# Autodesk Inventor assembly: Structure
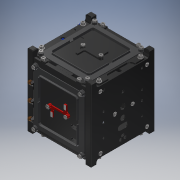
[picture p0: Inventor's stored thumbnail of the model, 180x180]
Saved by Autodesk Inventor 2018 (Build 220112000, 112)
## iProperties
Created: 2019-03-30
Part Number: Structure
Document SubType Name: Assembly
Designer: Bradley
Author: Bradley
## Documents named in this file (19)
- C:\Users\Bradley\Documents\GitHub\CougSat1-Hardware\CougSat1-Structure\CADModel\Imported\Structure.iam
- C:\Users\Bradley\Documents\GitHub\CougSat1-Hardware\CougSat1-Structure\CADModel\Imported\Structure_+X.ipt
- C:\Users\Bradley\Documents\GitHub\CougSat1-Hardware\CougSat1-Structure\CADModel\Imported\Structure_-X.ipt
- C:\Users\Bradley\Documents\GitHub\CougSat1-Hardware\CougSat1-Structure\CADModel\Imported\Structure_Y.ipt
- C:\Users\Bradley\Documents\GitHub\CougSat1-Hardware\CougSat1-Structure\CADModel\Imported\Structure_-Z.ipt
- C:\Users\Bradley\Documents\GitHub\CougSat1-Hardware\CougSat1-Structure\CADModel\Imported\Structure_SolarPanelHeatsink.ipt
- C:\Users\Bradley\Documents\GitHub\CougSat1-Hardware\CougSat1-Structure\CADModel\Imported\Structure_MagnetorquerForm.ipt
- C:\Users\Bradley\Documents\GitHub\Resources\SupplierDocuments\48 - Hardware\48-0361\48-0361.ipt
- C:\Users\Bradley\Documents\GitHub\Resources\SupplierDocuments\48 - Hardware\48-0340\48-0340.ipt
- C:\Users\Bradley\Documents\GitHub\Resources\SupplierDocuments\48 - Hardware\48-0350\48-0350.ipt
- C:\Users\Bradley\Documents\GitHub\Resources\SupplierDocuments\48 - Hardware\48-0300\48-0300.ipt
- C:\Users\Bradley\Documents\GitHub\Resources\SupplierDocuments\48 - Hardware\48-0001\48-0001.ipt
- C:\Users\Bradley\Documents\GitHub\Resources\SupplierDocuments\48 - Hardware\48-0381\48-0381.ipt
- C:\Users\Bradley\Documents\GitHub\Resources\SupplierDocuments\48 - Hardware\48-0362\48-0362.ipt
- C:\Users\Bradley\Documents\GitHub\Resources\SupplierDocuments\48 - Hardware\48-03A1\48-03A1.ipt
- C:\Users\Bradley\Documents\GitHub\Resources\SupplierDocuments\49 - Electromechanical\49-0006\49-0006.ipt
- C:\Users\Bradley\Documents\GitHub\CougSat1-Hardware\CougSat1-Payload\CADModel\Imported\Germination_Bottom.ipt
- C:\Users\Bradley\Documents\GitHub\CougSat1-Hardware\CougSat1-Payload\CADModel\Imported\Germination_Top.ipt
- C:\Users\Bradley\Documents\GitHub\Resources\SupplierDocuments\48 - Hardware\48-0280\48-0280.ipt
## Components (95 placed, 18 different names)
1. 48-0280:6 — Insert:143
2. 48-0280:5 — Insert:144
3. 48-0280:4 — Insert:145
4. 48-0280:3 — Insert:146
5. 48-0280:2 — Insert:147
6. 48-0280:1 — Insert:148
7. 48-0361:16 — Insert:101
8. 48-0361:15 — Insert:105
9. 48-0361:14 — Insert:104
10. 48-0361:13 — Insert:106
11. 48-0361:12 — Insert:103
12. 48-0361:11 — Insert:102
13. 48-0361:10 — Insert:100
14. 48-0361:9 — Insert:99
15. 49-0006:3 — Insert:138, Angle:3, Insert:143
16. 49-0006:2 — Insert:137, Angle:1, Insert:147
17. 49-0006:1 — Insert:139, Angle:2, Insert:145
18. 48-0001:1 — Insert:27
19. 48-0001:2 — Insert:140
20. 48-0300:1 — Insert:29, Insert:131
21. 48-0300:10 — Insert:129
22. 48-0300:11 — Insert:133
23. 48-0300:12 — Insert:54
24. 48-0300:2 — Insert:53
25. 48-0300:3 — Insert:51
26. 48-0300:4 — Insert:52
27. 48-0300:5 — Insert:83, Insert:87
28. 48-0300:6 — Insert:84, Insert:88
29. 48-0300:7 — Insert:85, Insert:90
30. 48-0300:8 — Insert:86, Insert:89
31. 48-0300:9 — Insert:136
32. 48-0340:1 — Insert:77
33. 48-0340:10 — Insert:90
34. 48-0340:2 — Insert:89
35. 48-0340:3 — Insert:78
36. 48-0340:4 — Insert:79
37. 48-0340:5 — Insert:80
38. 48-0340:6 — Insert:81
39. 48-0340:7 — Insert:82
40. 48-0340:8 — Insert:87
41. 48-0340:9 — Insert:88
42. 48-0350:1 — Insert:130
43. 48-0350:2 — Insert:132
44. 48-0350:3 — Insert:134
45. 48-0350:4 — Insert:135
46. 48-0350:5 — Insert:58
47. 48-0350:6 — Insert:57
48. 48-0350:7 — Insert:55
49. 48-0350:8 — Insert:56
50. 48-0362:1 — Insert:91
51. 48-0362:2 — Insert:92
52. 48-0362:3 — Insert:94
53. 48-0362:4 — Insert:93
54. 48-0361:1 — Insert:29
55. 48-0361:2
56. 48-0361:3
57. 48-0361:4
58. 48-0361:5
59. 48-0361:6
60. 48-0361:7
61. 48-0361:8
62. 48-0381:1 — Insert:59
63. 48-0381:18 — Insert:75
64. 48-0381:2 — Insert:60
65. 48-0381:3 — Insert:63
66. 48-0381:4 — Insert:64
67. 48-0381:5 — Insert:61
68. 48-0381:6 — Insert:62
69. 48-0381:7 — Insert:65
70. 48-0381:8 — Insert:66
71. 48-0381:9 — Insert:67
72. 48-0381:10 — Insert:68
73. 48-0381:11 — Insert:69
74. 48-0381:12 — Insert:70
75. 48-0381:13 — Insert:71
76. 48-0381:14 — Insert:72
77. 48-0381:15 — Insert:142
78. 48-0381:16 — Insert:141
79. 48-0381:17 — Insert:76
80. 48-03A1:1 — Insert:95
81. 48-03A1:2 — Insert:96
82. Germination_Top:1 — Insert:97, Insert:98, Insert:107, Insert:108, Insert:109, Insert:110, Insert:111, Insert:112, Insert:113, Insert:114, Insert:115, Insert:116, Insert:129, Insert:130, Insert:131, Insert:132, Insert:133, Insert:134, Insert:135, Insert:136, Insert:141, Insert:142
83. Germination_Bottom:1 — Insert:97, Insert:98, Insert:99, Insert:100, Insert:101, Insert:102, Insert:103, Insert:104, Insert:105, Insert:106
84. Structure_+X:1 — Mate:1, Mate:2, Mate:3, Insert:9, Insert:10, Insert:27, Insert:77, Insert:78, Insert:79, Insert:80, Insert:81, Insert:82, Insert:107, Insert:108
85. Structure_-X:1 — Insert:113, Insert:114, Insert:119, Insert:120, Insert:127, Insert:128, Insert:137, Insert:138, Insert:139, Angle:1, Angle:2, Angle:3, Insert:140, Insert:144, Insert:146, Insert:148
86. Structure_-Z:1 — Insert:9, Insert:10, Insert:51, Insert:52, Insert:53, Insert:54, Insert:55, Insert:56, Insert:57, Insert:58, Insert:83, Insert:84, Insert:85, Insert:86
87. Structure_MagnetorquerForm:1 — Insert:59, Insert:60, Insert:63, Insert:64, Insert:117, Insert:118
88. Structure_MagnetorquerForm:2 — Insert:91, Insert:92, Insert:93, Insert:94, Insert:119, Insert:120
89. Structure_MagnetorquerForm:3 — Insert:71, Insert:72, Insert:75, Insert:76, Insert:115, Insert:116
90. Structure_MagnetorquerForm:4 — Insert:65, Insert:66, Insert:69, Insert:70, Insert:121, Insert:122
91. Structure_SolarPanelHeatsink:2 — Insert:61, Insert:62, Insert:125, Insert:126
92. Structure_SolarPanelHeatsink:3 — Insert:95, Insert:96, Insert:127, Insert:128
93. Structure_SolarPanelHeatsink:4 — Insert:67, Insert:68, Insert:123, Insert:124
94. Structure_Y:1 — Insert:111, Insert:112, Insert:117, Insert:118, Insert:125, Insert:126
95. Structure_Y:2 — Insert:109, Insert:110, Insert:121, Insert:122, Insert:123, Insert:124
## Relationships (113: Insert 107, Mate 3, Angle 3)
- Mate:1 (50 mm): Structure_+X:1
- Mate:2 (-49 mm): Structure_+X:1
- Mate:3 (50 mm): Structure_+X:1
- Insert:9: Structure_+X:1 ↔ Structure_-Z:1
- Insert:10: Structure_+X:1 ↔ Structure_-Z:1
- Insert:27: 48-0001:1 ↔ Structure_+X:1
- Insert:29: 48-0300:1 ↔ 48-0361:1
- [Insert]: 48-0300:9 ↔ 48-0361:5
- [Insert]: 48-0300:10 ↔ 48-0361:6
- [Insert]: 48-0300:11 ↔ 48-0361:7
- [Insert]: 48-0300:12 ↔ 48-0361:8
- [Insert]: 48-0300:2 ↔ 48-0361:2
- [Insert]: 48-0300:3 ↔ 48-0361:3
- [Insert]: 48-0300:4 ↔ 48-0361:4
- Insert:51: 48-0300:3 ↔ Structure_-Z:1
- Insert:52: 48-0300:4 ↔ Structure_-Z:1
- Insert:53: 48-0300:2 ↔ Structure_-Z:1
- Insert:54: 48-0300:12 ↔ Structure_-Z:1
- Insert:55: 48-0350:7 ↔ Structure_-Z:1
- Insert:56: 48-0350:8 ↔ Structure_-Z:1
- Insert:57: 48-0350:6 ↔ Structure_-Z:1
- Insert:58: 48-0350:5 ↔ Structure_-Z:1
- Insert:59 (1 mm): 48-0381:1 ↔ Structure_MagnetorquerForm:1
- Insert:60 (1 mm): 48-0381:2 ↔ Structure_MagnetorquerForm:1
- Insert:61 (1 mm): 48-0381:5 ↔ Structure_SolarPanelHeatsink:2
- Insert:62 (1 mm): 48-0381:6 ↔ Structure_SolarPanelHeatsink:2
- Insert:63 (1 mm): 48-0381:3 ↔ Structure_MagnetorquerForm:1
- Insert:64 (1 mm): 48-0381:4 ↔ Structure_MagnetorquerForm:1
- Insert:65 (1 mm): 48-0381:7 ↔ Structure_MagnetorquerForm:4
- Insert:66 (1 mm): 48-0381:8 ↔ Structure_MagnetorquerForm:4
- Insert:67 (1 mm): 48-0381:9 ↔ Structure_SolarPanelHeatsink:4
- Insert:68 (1 mm): 48-0381:10 ↔ Structure_SolarPanelHeatsink:4
- Insert:69 (1 mm): 48-0381:11 ↔ Structure_MagnetorquerForm:4
- Insert:70 (1 mm): 48-0381:12 ↔ Structure_MagnetorquerForm:4
- Insert:71 (1 mm): 48-0381:13 ↔ Structure_MagnetorquerForm:3
- Insert:72 (1 mm): 48-0381:14 ↔ Structure_MagnetorquerForm:3
- Insert:75 (1 mm): 48-0381:18 ↔ Structure_MagnetorquerForm:3
- Insert:76 (1 mm): 48-0381:17 ↔ Structure_MagnetorquerForm:3
- Insert:77 (1 mm): 48-0340:1 ↔ Structure_+X:1
- Insert:78 (1 mm): 48-0340:3 ↔ Structure_+X:1
- Insert:79 (1 mm): 48-0340:4 ↔ Structure_+X:1
- Insert:80 (1 mm): 48-0340:5 ↔ Structure_+X:1
- Insert:81 (1 mm): 48-0340:6 ↔ Structure_+X:1
- Insert:82 (1 mm): 48-0340:7 ↔ Structure_+X:1
- Insert:83: 48-0300:5 ↔ Structure_-Z:1
- Insert:84: 48-0300:6 ↔ Structure_-Z:1
- Insert:85: 48-0300:7 ↔ Structure_-Z:1
- Insert:86: 48-0300:8 ↔ Structure_-Z:1
- Insert:87 (1 mm): 48-0300:5 ↔ 48-0340:8
- Insert:88 (1 mm): 48-0300:6 ↔ 48-0340:9
- Insert:89 (1 mm): 48-0300:8 ↔ 48-0340:2
- Insert:90 (1 mm): 48-0300:7 ↔ 48-0340:10
- Insert:91 (1 mm): 48-0362:1 ↔ Structure_MagnetorquerForm:2
- Insert:92 (1 mm): 48-0362:2 ↔ Structure_MagnetorquerForm:2
- Insert:93 (1 mm): 48-0362:4 ↔ Structure_MagnetorquerForm:2
- Insert:94 (1 mm): 48-0362:3 ↔ Structure_MagnetorquerForm:2
- Insert:95 (1 mm): 48-03A1:1 ↔ Structure_SolarPanelHeatsink:3
- Insert:96 (1 mm): 48-03A1:2 ↔ Structure_SolarPanelHeatsink:3
- Insert:97: Germination_Top:1 ↔ Germination_Bottom:1
- Insert:98: Germination_Top:1 ↔ Germination_Bottom:1
- Insert:99: 48-0361:9 ↔ Germination_Bottom:1
- Insert:100: 48-0361:10 ↔ Germination_Bottom:1
- Insert:101: 48-0361:16 ↔ Germination_Bottom:1
- Insert:102: 48-0361:11 ↔ Germination_Bottom:1
- Insert:103: 48-0361:12 ↔ Germination_Bottom:1
- Insert:104: 48-0361:14 ↔ Germination_Bottom:1
- Insert:105: 48-0361:15 ↔ Germination_Bottom:1
- Insert:106: 48-0361:13 ↔ Germination_Bottom:1
- Insert:107: Germination_Top:1 ↔ Structure_+X:1
- Insert:108: Germination_Top:1 ↔ Structure_+X:1
- Insert:109: Germination_Top:1 ↔ Structure_Y:2
- Insert:110: Germination_Top:1 ↔ Structure_Y:2
- Insert:111: Germination_Top:1 ↔ Structure_Y:1
- Insert:112: Germination_Top:1 ↔ Structure_Y:1
- Insert:113: Germination_Top:1 ↔ Structure_-X:1
- Insert:114: Germination_Top:1 ↔ Structure_-X:1
- Insert:115: Germination_Top:1 ↔ Structure_MagnetorquerForm:3
- Insert:116: Germination_Top:1 ↔ Structure_MagnetorquerForm:3
- Insert:117: Structure_MagnetorquerForm:1 ↔ Structure_Y:1
- Insert:118: Structure_MagnetorquerForm:1 ↔ Structure_Y:1
- Insert:119: Structure_-X:1 ↔ Structure_MagnetorquerForm:2
- Insert:120: Structure_-X:1 ↔ Structure_MagnetorquerForm:2
- Insert:121: Structure_MagnetorquerForm:4 ↔ Structure_Y:2
- Insert:122: Structure_MagnetorquerForm:4 ↔ Structure_Y:2
- Insert:123: Structure_SolarPanelHeatsink:4 ↔ Structure_Y:2
- Insert:124: Structure_SolarPanelHeatsink:4 ↔ Structure_Y:2
- Insert:125: Structure_SolarPanelHeatsink:2 ↔ Structure_Y:1
- Insert:126: Structure_SolarPanelHeatsink:2 ↔ Structure_Y:1
- Insert:127: Structure_-X:1 ↔ Structure_SolarPanelHeatsink:3
- Insert:128: Structure_-X:1 ↔ Structure_SolarPanelHeatsink:3
- Insert:129: 48-0300:10 ↔ Germination_Top:1
- Insert:130: 48-0350:1 ↔ Germination_Top:1
- Insert:131: 48-0300:1 ↔ Germination_Top:1
- Insert:132: 48-0350:2 ↔ Germination_Top:1
- Insert:133: 48-0300:11 ↔ Germination_Top:1
- Insert:134: 48-0350:3 ↔ Germination_Top:1
- Insert:135: 48-0350:4 ↔ Germination_Top:1
- Insert:136: 48-0300:9 ↔ Germination_Top:1
- Insert:137: 49-0006:2 ↔ Structure_-X:1
- Insert:138: 49-0006:3 ↔ Structure_-X:1
- Insert:139: 49-0006:1 ↔ Structure_-X:1
- Angle:1 (0 deg): 49-0006:2 ↔ Structure_-X:1
- Angle:2 (0 deg): 49-0006:1 ↔ Structure_-X:1
- Angle:3 (0 deg): 49-0006:3 ↔ Structure_-X:1
- Insert:140: 48-0001:2 ↔ Structure_-X:1
- Insert:141 (1 mm): 48-0381:16 ↔ Germination_Top:1
- Insert:142 (1 mm): 48-0381:15 ↔ Germination_Top:1
- Insert:143: 48-0280:6 ↔ 49-0006:3
- Insert:144 (6.4 mm): 48-0280:5 ↔ Structure_-X:1
- Insert:145: 48-0280:4 ↔ 49-0006:1
- Insert:146 (6.4 mm): 48-0280:3 ↔ Structure_-X:1
- Insert:147: 48-0280:2 ↔ 49-0006:2
- Insert:148 (6.4 mm): 48-0280:1 ↔ Structure_-X:1
## Named parameters: d36_d32 = 0 mm, d37_d32 = 0 mm, d40_d32 = 0 mm, d52_d32 = 0 mm, d53_d32 = 0 mm, d54_d32 = 0 mm, d55_d32 = 0 mm, SolarPanelThickness = 1 mm, PXThickness = 1 mm, NZThickness = 1 mm
